# Autodesk Inventor assembly: esp32-faerfly-case-V2.0
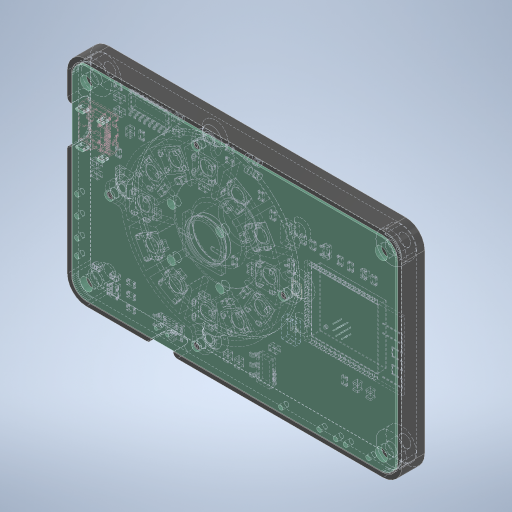
[picture p0: Inventor's stored thumbnail of the model, 512x512]
Saved by Autodesk Inventor 2023 (Build 270158030, 158C)
## iProperties
Created: 2023-04-27
Part Number: esp32-faerfly-case-V2.0
Document SubType Name: Assembly
Designer: Imogen Heard
Author: Imogen Heard
## Documents named in this file (4)
- C:\Users\dheard\Documents\0000.KiCad\Projects\000-personal-projects\esp32-faerfly\3D-cad\esp32-faerfly-inventor\esp32-faerfly-case-V2.0.iam
- C:\Users\dheard\Documents\0000.KiCad\Projects\000-personal-projects\esp32-faerfly\3D-cad\esp32-faerfly-model.ipt
- C:\Users\dheard\Documents\0000.KiCad\Projects\000-personal-projects\esp32-faerfly\3D-cad\esp32-faerfly-inventor\case-topside-V2.0.ipt
- C:\Users\dheard\Documents\0000.KiCad\Projects\000-personal-projects\esp32-faerfly\3D-cad\esp32-faerfly-inventor\case-stls\V2.0-case-outer-cover.ipt
## Components (3 placed, 3 different names)
1. esp32-faerfly-model:1 — Flush:1, Flush:2
2. case-topside-V2.0:1 — Flush:1, Flush:2, Flush:3, Flush:4
3. V2.0-case-outer-cover:1 — Flush:3, Flush:4
## Relationships (4: Flush 4)
- Flush:1: esp32-faerfly-model:1 ↔ case-topside-V2.0:1
- Flush:2: esp32-faerfly-model:1 ↔ case-topside-V2.0:1
- Flush:3: case-topside-V2.0:1 ↔ V2.0-case-outer-cover:1
- Flush:4: case-topside-V2.0:1 ↔ V2.0-case-outer-cover:1
